# Autodesk Inventor assembly: simplified
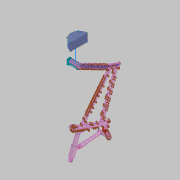
[picture p0: Inventor's stored thumbnail of the model, 180x180]
Saved by Autodesk Inventor 2021 (Build 250183000, 183)
## iProperties
Created: 2020-05-04
Part Number: simplified
Document SubType Name: Assembly
Designer: Hannah
Author: Hannah
## Documents named in this file (5)
- \\Mac\Home\Documents\GitHub\AdjustaBike-2.0\CAD\simplified.iam
- \\Mac\Home\Documents\GitHub\AdjustaBike-2.0\CAD\Solid3_1.ipt
- \\Mac\Home\Documents\GitHub\AdjustaBike-2.0\CAD\Solid4_1.ipt
- \\Mac\Home\Documents\GitHub\AdjustaBike-2.0\CAD\Solid5_1.ipt
- \\Mac\Home\Documents\GitHub\AdjustaBike-2.0\CAD\projectile.ipt
## Components (4 placed, 4 different names)
1. Solid3_1:1
2. Solid4_1:1
3. Solid5_1:1 — Tangent:1, Mate:1
4. projectile:1 — Tangent:1, Angle:1, Mate:1, Flush:3
## Relationships (5: Flush 2, Tangent 1, Angle 1, Mate 1)
- Tangent:1 (180 mm): Solid5_1:1 ↔ projectile:1
- Angle:1 (0 deg): projectile:1
- Mate:1: Solid5_1:1 ↔ projectile:1
- Flush:3: projectile:1
- Flush:4 (-50 mm)
